# Autodesk Inventor assembly: Catapulta
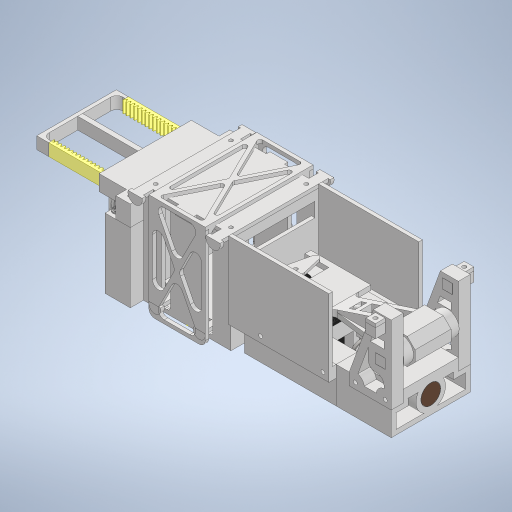
[picture p0: Inventor's stored thumbnail of the model, 512x512]
Saved by Autodesk Inventor 2024 (Build 280153000, 153)
## iProperties
Created: 2025-03-01
Part Number: Catapulta
Document SubType Name: Assembly
Designer: sergi
Author: sergi
## Documents named in this file (16)
- C:\Users\sergi\OneDrive\Escritorio\GitHub\16. Catapult\Inventor\Catapulta.iam
- C:\Users\sergi\OneDrive\Escritorio\GitHub\16. Catapult\Inventor\Base Catapulta.ipt
- C:\Users\sergi\OneDrive\Escritorio\GitHub\16. Catapult\Inventor\motor2.ipt
- C:\Users\sergi\OneDrive\Escritorio\GitHub\16. Catapult\Inventor\Acople motor.ipt
- C:\Users\sergi\OneDrive\Escritorio\GitHub\16. Catapult\Inventor\Polea.ipt
- C:\Users\sergi\OneDrive\Escritorio\GitHub\16. Catapult\Inventor\Brazo.ipt
- C:\Users\sergi\OneDrive\Escritorio\GitHub\16. Catapult\Inventor\ServoMotor.ipt
- C:\Users\sergi\OneDrive\Escritorio\GitHub\16. Catapult\Inventor\Soporte lateral.ipt
- C:\Users\sergi\OneDrive\Escritorio\GitHub\16. Catapult\Inventor\Refuerzo superior.ipt
- C:\Users\sergi\OneDrive\Escritorio\GitHub\16. Catapult\Inventor\Refuerzo bisagra.ipt
- C:\Users\sergi\OneDrive\Escritorio\GitHub\16. Catapult\Inventor\Soporte gomas.ipt
- C:\Users\sergi\OneDrive\Escritorio\GitHub\16. Catapult\Inventor\Brazo catapulta.ipt
- C:\Users\sergi\OneDrive\Escritorio\GitHub\16. Catapult\Inventor\Adaptador servo.ipt
- C:\Users\sergi\OneDrive\Escritorio\GitHub\16. Catapult\Inventor\Tolva.iam
- C:\Users\sergi\OneDrive\Escritorio\GitHub\16. Catapult\Inventor\Dispensador.iam
- C:\Users\sergi\OneDrive\Escritorio\GitHub\16. Catapult\Inventor\Separadores.ipt
## Components (19 placed, 15 different names)
1. Base Catapulta:1 — Nivelación:1, Coincidencia:6, Ángulo:1, Coincidencia:7, Ángulo:2, Coincidencia:11, Coincidencia:12, Ángulo:3, Coincidencia:24, Coincidencia:25, Nivelación:19, Nivelación:20
2. motor2:1 — Coincidencia:1, Coincidencia:2, Nivelación:1, Coincidencia:6, Ángulo:1
3. Acople motor:1 — Coincidencia:1, Coincidencia:2, Coincidencia:4, Coincidencia:5, Coincidencia:35
4. Polea:1 — Coincidencia:4, Coincidencia:5, Coincidencia:35
5. Brazo:1 — Coincidencia:8, Coincidencia:9, Ángulo:2
6. ServoMotor:1 — Coincidencia:7, Coincidencia:8, Coincidencia:9, Coincidencia:24, Coincidencia:25
7. Soporte lateral:1 — Coincidencia:11, Coincidencia:13, Coincidencia:14, Nivelación:9, Nivelación:18, Coincidencia:21, Nivelación:13
8. Soporte lateral:2 — Coincidencia:12, Nivelación:8, Nivelación:10, Coincidencia:19, Coincidencia:22, Nivelación:14, Coincidencia:23, Coincidencia:15, Coincidencia:16
9. Refuerzo superior:1 — Coincidencia:13, Coincidencia:14, Nivelación:8, Nivelación:18, Nivelación:11, Coincidencia:18, Nivelación:12, Nivelación:13, Coincidencia:31
10. Refuerzo bisagra:1 — Nivelación:9, Coincidencia:15, Coincidencia:16, Nivelación:10, Coincidencia:20, Coincidencia:32, Coincidencia:34
11. Soporte gomas:1 — Nivelación:11, Coincidencia:31
12. Soporte gomas:2 — Coincidencia:18, Coincidencia:19, Nivelación:12
13. Brazo catapulta:1 — Coincidencia:20, Coincidencia:21, Ángulo:3, Nivelación:22, Coincidencia:33
14. Refuerzo superior:2 — Coincidencia:22, Nivelación:14, Coincidencia:23
15. Adaptador servo:1 — Nivelación:19, Coincidencia:26, Coincidencia:27, Nivelación:20, Nivelación:21, Coincidencia:28, Coincidencia:29, Coincidencia:30
16. Tolva:1 [sub-assembly] — Coincidencia:28, Coincidencia:29, Coincidencia:30
17. Dispensador:1 [sub-assembly] — Coincidencia:26, Coincidencia:27, Nivelación:21
18. Separadores:1 — Nivelación:22, Coincidencia:32
19. Separadores:2 — Coincidencia:33, Coincidencia:34
## Relationships (52: Mate 32, Flush 17, Angle 3)
- Coincidencia:1 [Mate]: motor2:1 ↔ Acople motor:1
- Coincidencia:2 [Mate]: motor2:1 ↔ Acople motor:1
- Coincidencia:4 [Mate]: Acople motor:1 ↔ Polea:1
- Coincidencia:5 [Mate]: Acople motor:1 ↔ Polea:1
- Nivelación:1 [Flush]: Base Catapulta:1 ↔ motor2:1
- Coincidencia:6 [Mate]: Base Catapulta:1 ↔ motor2:1
- Ángulo:1 [Angle] (0 deg): Base Catapulta:1 ↔ motor2:1
- Coincidencia:7 [Mate]: Base Catapulta:1 ↔ ServoMotor:1
- Coincidencia:8 [Mate]: Brazo:1 ↔ ServoMotor:1
- Coincidencia:9 [Mate]: Brazo:1 ↔ ServoMotor:1
- Ángulo:2 [Angle] (0 deg): Base Catapulta:1 ↔ Brazo:1
- Coincidencia:11 [Mate]: Base Catapulta:1 ↔ Soporte lateral:1
- [Flush]: Base Catapulta:1 ↔ Soporte lateral:1
- [Flush]: Base Catapulta:1 ↔ Soporte lateral:1
- [Flush]: Base Catapulta:1 ↔ Soporte lateral:2
- [Flush]: Base Catapulta:1 ↔ Soporte lateral:2
- Coincidencia:12 [Mate]: Base Catapulta:1 ↔ Soporte lateral:2
- Coincidencia:13 [Mate] (0.1 mm): Soporte lateral:1 ↔ Refuerzo superior:1
- Coincidencia:14 [Mate] (0.1 mm): Soporte lateral:1 ↔ Refuerzo superior:1
- Nivelación:8 [Flush]: Soporte lateral:2 ↔ Refuerzo superior:1
- Nivelación:9 [Flush]: Soporte lateral:1 ↔ Refuerzo bisagra:1
- Coincidencia:15 [Mate] (0.1 mm): Soporte lateral:2 ↔ Refuerzo bisagra:1
- Coincidencia:16 [Mate] (0.1 mm): Soporte lateral:2 ↔ Refuerzo bisagra:1
- Nivelación:10 [Flush]: Soporte lateral:2 ↔ Refuerzo bisagra:1
- Nivelación:18 [Flush]: Soporte lateral:1 ↔ Refuerzo superior:1
- Nivelación:11 [Flush]: Refuerzo superior:1 ↔ Soporte gomas:1
- Coincidencia:18 [Mate]: Refuerzo superior:1 ↔ Soporte gomas:2
- Coincidencia:19 [Mate]: Soporte lateral:2 ↔ Soporte gomas:2
- Nivelación:12 [Flush]: Refuerzo superior:1 ↔ Soporte gomas:2
- Coincidencia:20 [Mate]: Refuerzo bisagra:1 ↔ Brazo catapulta:1
- Coincidencia:21 [Mate] (8 mm): Soporte lateral:1 ↔ Brazo catapulta:1
- Ángulo:3 [Angle] (-180 deg): Base Catapulta:1 ↔ Brazo catapulta:1
- Nivelación:13 [Flush]: Soporte lateral:1 ↔ Refuerzo superior:1
- Coincidencia:22 [Mate] (0.1 mm): Soporte lateral:2 ↔ Refuerzo superior:2
- Nivelación:14 [Flush]: Soporte lateral:2 ↔ Refuerzo superior:2
- Coincidencia:23 [Mate] (0.1 mm): Soporte lateral:2 ↔ Refuerzo superior:2
- Coincidencia:24 [Mate]: Base Catapulta:1 ↔ ServoMotor:1
- Coincidencia:25 [Mate] (36 mm): Base Catapulta:1 ↔ ServoMotor:1
- Nivelación:19 [Flush]: Base Catapulta:1 ↔ Adaptador servo:1
- Coincidencia:26 [Mate]: Adaptador servo:1 ↔ Dispensador:1
- Coincidencia:27 [Mate]: Adaptador servo:1 ↔ Dispensador:1
- Nivelación:20 [Flush]: Base Catapulta:1 ↔ Adaptador servo:1
- Nivelación:21 [Flush]: Adaptador servo:1 ↔ Dispensador:1
- Coincidencia:28 [Mate]: Adaptador servo:1 ↔ Tolva:1
- Coincidencia:29 [Mate]: Adaptador servo:1 ↔ Tolva:1
- Coincidencia:30 [Mate]: Adaptador servo:1 ↔ Tolva:1
- Coincidencia:31 [Mate]: Refuerzo superior:1 ↔ Soporte gomas:1
- Nivelación:22 [Flush]: Brazo catapulta:1 ↔ Separadores:1
- Coincidencia:32 [Mate]: Refuerzo bisagra:1 ↔ Separadores:1
- Coincidencia:33 [Mate]: Brazo catapulta:1 ↔ Separadores:2
- Coincidencia:34 [Mate]: Refuerzo bisagra:1 ↔ Separadores:2
- Coincidencia:35 [Mate]: Acople motor:1 ↔ Polea:1
